# Autodesk Inventor assembly: Output Link
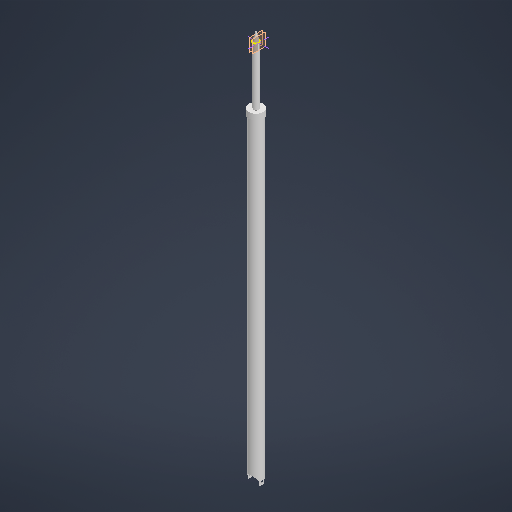
[picture p0: Inventor's stored thumbnail of the model, 512x512]
Saved by Autodesk Inventor 2026.3 (Build 303398000, 398)
## iProperties
Created: 2026-07-24
Part Number: Output Link
Document SubType Name: Assembly
Designer: matot
Author: matot
## Documents named in this file (6)
- C:\Users\matot\OneDrive - Stellenbosch University\2026\MechatronicsProject478\Building the joint\Joint Assembly\Output Link.iam
- C:\Users\matot\OneDrive - Stellenbosch University\2026\MechatronicsProject478\Building the joint\Joint Assembly\Output link probe.ipt
- C:\Users\matot\OneDrive - Stellenbosch University\2026\MechatronicsProject478\Building the joint\Joint Assembly\Output link body_ final.ipt
- C:\Users\matot\OneDrive - Stellenbosch University\2026\MechatronicsProject478\Building the joint\Joint Assembly\Output link probe hub_ final.ipt
- C:\Users\matot\OneDrive - Stellenbosch University\2026\MechatronicsProject478\Building the joint\Joint Assembly\Washer ID 10.ipt
- C:\Users\matot\OneDrive - Stellenbosch University\2026\MechatronicsProject478\Building the joint\Joint Assembly\M10x1.5 Nut.ipt
## Components (5 placed, 5 different names)
1. Output link body_ final:1 — Insert:4
2. Output link probe hub_ final:1 — Insert:1, Insert:2, Insert:4
3. Output link probe:1 — Insert:1
4. Washer ID 10:2 — Insert:2, Insert:3
5. M10x1.5 Nut:2 — Insert:3
## Relationships (4: Insert 4)
- Insert:1 (-40 mm): Output link probe hub_ final:1 ↔ Output link probe:1
- Insert:2: Output link probe hub_ final:1 ↔ Washer ID 10:2
- Insert:3: Washer ID 10:2 ↔ M10x1.5 Nut:2
- Insert:4: Output link body_ final:1 ↔ Output link probe hub_ final:1
